# Autodesk Inventor assembly: Assembly_cellSTORM_inverted_opticmodule_v0
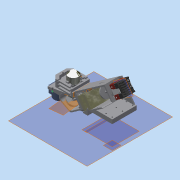
[picture p0: Inventor's stored thumbnail of the model, 180x180]
Saved by Autodesk Inventor 2019.4 (Build 234330000, 330)
## iProperties
Created: 2020-11-06
Part Number: Assembly_cellSTORM_inverted_opticmodule_v0
Document SubType Name: Assembly
Designer: diederichbenedict
Author: diederichbenedict
## Documents named in this file (13)
- C:\Users\diederichbenedict\Dropbox\Dokumente\Promotion\PROJECTS\STORMoChip\GITHUB\CAD\cellSTORM_inverted\Workspace\Assembly_cellSTORM_inverted_opticmodule_v0.iam
- C:\Users\diederichbenedict\Dropbox\Dokumente\Promotion\PROJECTS\STORMoChip\GITHUB\CAD\cellSTORM_inverted\Workspace\00_Microscope_Objective.ipt
- C:\Users\diederichbenedict\Dropbox\Dokumente\Promotion\PROJECTS\STORMoChip\GITHUB\CAD\cellSTORM_inverted\Workspace\cellSTORM_lightpath.ipt
- C:\Users\diederichbenedict\Dropbox\Dokumente\Promotion\PROJECTS\STORMoChip\GITHUB\CAD\cellSTORM_inverted\Workspace\PF10-03-P01-Step.ipt
- C:\Users\diederichbenedict\Dropbox\Dokumente\Promotion\PROJECTS\STORMoChip\GITHUB\CAD\cellSTORM_inverted\Workspace\00_Alvium_Step_USB90_S-Mount_ClosedHousing_2019-Mar-28.ipt
- C:\Users\diederichbenedict\Dropbox\Dokumente\Promotion\PROJECTS\STORMoChip\GITHUB\CAD\cellSTORM_inverted\Workspace\AC254-050-A-ML-Step.ipt
- C:\Users\diederichbenedict\Dropbox\Dokumente\Promotion\PROJECTS\STORMoChip\GITHUB\CAD\cellSTORM_inverted\Workspace\10_Filteslide_25mm.ipt
- C:\Users\diederichbenedict\Dropbox\Dokumente\Promotion\PROJECTS\STORMoChip\GITHUB\CAD\cellSTORM_inverted\Workspace\cellSTORM_inverted_opticsmodule_v0.ipt
- C:\Users\diederichbenedict\Dropbox\Dokumente\Promotion\PROJECTS\STORMoChip\GITHUB\CAD\cellSTORM_inverted\Workspace\00_Stepper_Motor_28BYJ-48.0013.ipt
- C:\Users\diederichbenedict\Dropbox\Dokumente\Promotion\PROJECTS\STORMoChip\GITHUB\CAD\cellSTORM_inverted\Workspace\cellSTORM_inverted_opticsmodule_lid.ipt
- C:\Users\diederichbenedict\Dropbox\Dokumente\Promotion\PROJECTS\STORMoChip\GITHUB\CAD\cellSTORM_inverted\Workspace\cellSTORM_v5_focussingunit_1.ipt
- C:\Users\diederichbenedict\Dropbox\Dokumente\Promotion\PROJECTS\STORMoChip\GITHUB\CAD\cellSTORM_inverted\Workspace\cellSTORM_inverted_objectiveadapter.ipt
- C:\Users\diederichbenedict\Dropbox\Dokumente\Promotion\PROJECTS\STORMoChip\GITHUB\CAD\cellSTORM_inverted\Workspace\cellSTORM_Alvium_cameraadapter.ipt
## Components (13 placed, 12 different names)
1. 00_Microscope_Objective:1
2. PF10-03-P01-Step:1
3. 00_Stepper_Motor_28BYJ-48.0013:1
4. cellSTORM_lightpath:1 — Mate:10, Mate:11
5. cellSTORM_inverted_opticsmodule_v0:1 — Flush:1, Angle:4, Angle:5, Insert:8
6. cellSTORM_v5_focussingunit_1:1 — Flush:6
7. cellSTORM_inverted_objectiveadapter:1 — Flush:6
8. cellSTORM_inverted_opticsmodule_lid:1
9. AC254-050-A-ML-Step:1 — Insert:7, Mate:11
10. 10_Filteslide_25mm:2 — Mate:10, Angle:5
11. 10_Filteslide_25mm:3 — Insert:7, Angle:4
12. 00_Alvium_Step_USB90_S-Mount_ClosedHousing_2019-Mar-28:1 — Insert:8, Flush:7, Flush:8
13. cellSTORM_Alvium_cameraadapter:1 — Flush:7, Flush:8
## Relationships (13: Insert 5, Flush 4, Mate 2, Angle 2)
- [Insert]: PF10-03-P01-Step:1 ↔ cellSTORM_lightpath:1
- [Insert]: 00_Microscope_Objective:1 ↔ cellSTORM_lightpath:1
- Flush:1: cellSTORM_inverted_opticsmodule_v0:1
- [Insert]: cellSTORM_inverted_opticsmodule_v0:1 ↔ cellSTORM_v5_focussingunit_1:1
- Flush:6: cellSTORM_v5_focussingunit_1:1 ↔ cellSTORM_inverted_objectiveadapter:1
- Mate:10: cellSTORM_lightpath:1 ↔ 10_Filteslide_25mm:2
- Insert:7: AC254-050-A-ML-Step:1 ↔ 10_Filteslide_25mm:3
- Angle:4 (0 deg): cellSTORM_inverted_opticsmodule_v0:1 ↔ 10_Filteslide_25mm:3
- Mate:11: cellSTORM_lightpath:1 ↔ AC254-050-A-ML-Step:1
- Angle:5 (0 deg): cellSTORM_inverted_opticsmodule_v0:1 ↔ 10_Filteslide_25mm:2
- Insert:8 (4 mm): cellSTORM_inverted_opticsmodule_v0:1 ↔ 00_Alvium_Step_USB90_S-Mount_ClosedHousing_2019-Mar-28:1
- Flush:7: 00_Alvium_Step_USB90_S-Mount_ClosedHousing_2019-Mar-28:1 ↔ cellSTORM_Alvium_cameraadapter:1
- Flush:8: 00_Alvium_Step_USB90_S-Mount_ClosedHousing_2019-Mar-28:1 ↔ cellSTORM_Alvium_cameraadapter:1
